# Autodesk Inventor assembly: PMax8
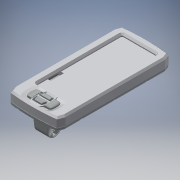
[picture p0: Inventor's stored thumbnail of the model, 180x180]
Saved by Autodesk Inventor 2018 (Build 220112000, 112)
## iProperties
Created: 2019-05-29
Part Number: PMax8
Document SubType Name: Assembly
Designer: Ash
Author: Ash
## Documents named in this file (8)
- C:\Autodesk\Skills 2019 Nationals\Competition\PMDay2\PMax8.iam
- C:\Autodesk\Skills 2019 Nationals\Competition\PMDay2\#2-KEYPAD.ipt
- C:\Autodesk\Skills 2019 Nationals\Competition\PMDay1\Front_Cover3.ipt
- C:\Autodesk\Skills 2019 Nationals\Competition\PMDay1\Display_Plate3.ipt
- C:\Autodesk\Skills 2019 Nationals\Competition\PMDay2\#4-GASKET(PMAX8).ipt
- C:\Autodesk\Skills 2019 Nationals\Competition\PMDay2\#5-BACK_COVER(PMAX8).ipt
- C:\Autodesk\Skills 2019 Nationals\Competition\PMDay2\ADDITIONAL_BUTTON.ipt
- C:\Autodesk\Skills 2019 Nationals\Competition\PMDay2\#6-SCREW.ipt
## Components (16 placed, 7 different names)
1. #2-KEYPAD:1 — Mate:6, Mate:7, Mate:8, Mate:9, Mate:11
2. Display_Plate3:1 — Mate:7, Mate:10, Mate:11
3. Front_Cover3:1 — Mate:6, Mate:8, Mate:9, Mate:10, Mate:15, Mate:16, Mate:17, Mate:18, Flush:1
4. #4-GASKET(PMAX8):1 — Mate:12, Mate:13, Mate:14, Mate:19
5. #5-BACK_COVER(PMAX8):1 — Mate:12, Mate:13, Mate:14, Mate:15, Mate:16, Mate:17, Mate:20, Mate:21, Mate:22, Mate:23, Mate:24, Mate:25, Mate:26, Mate:27, Mate:28, Mate:29, Mate:30
6. ADDITIONAL_BUTTON:1 — Mate:18, Mate:19, Flush:1
7. #6-SCREW:1 — Mate:28, Flush:2
8. #6-SCREW:2 — Mate:22, Flush:9, Flush:10
9. #6-SCREW:3 — Mate:21, Flush:8, Flush:9, Mate:30
10. #6-SCREW:4 — Mate:29, Flush:10
11. #6-SCREW:5 — Mate:23, Flush:6, Flush:7
12. #6-SCREW:6 — Mate:27, Flush:2, Flush:3
13. #6-SCREW:7 — Mate:26, Flush:3, Flush:4
14. #6-SCREW:8 — Mate:24, Flush:5, Flush:6
15. #6-SCREW:9 — Mate:25, Flush:4, Flush:5
16. #6-SCREW:10 — Mate:20, Flush:7, Flush:8
## Relationships (35: Mate 25, Flush 10)
- Mate:6 (6.35 mm): #2-KEYPAD:1 ↔ Front_Cover3:1
- Mate:7: #2-KEYPAD:1 ↔ Display_Plate3:1
- Mate:8: #2-KEYPAD:1 ↔ Front_Cover3:1
- Mate:9 (46.7868 mm): #2-KEYPAD:1 ↔ Front_Cover3:1
- Mate:10: Display_Plate3:1 ↔ Front_Cover3:1
- Mate:11: #2-KEYPAD:1 ↔ Display_Plate3:1
- Mate:12: #4-GASKET(PMAX8):1 ↔ #5-BACK_COVER(PMAX8):1
- Mate:13: #4-GASKET(PMAX8):1 ↔ #5-BACK_COVER(PMAX8):1
- Mate:14: #4-GASKET(PMAX8):1 ↔ #5-BACK_COVER(PMAX8):1
- Mate:15: Front_Cover3:1 ↔ #5-BACK_COVER(PMAX8):1
- Mate:16: Front_Cover3:1 ↔ #5-BACK_COVER(PMAX8):1
- Mate:17: Front_Cover3:1 ↔ #5-BACK_COVER(PMAX8):1
- Mate:18 (-10.16 mm): Front_Cover3:1 ↔ ADDITIONAL_BUTTON:1
- Mate:19 (6.35 mm): #4-GASKET(PMAX8):1 ↔ ADDITIONAL_BUTTON:1
- Flush:1: Front_Cover3:1 ↔ ADDITIONAL_BUTTON:1
- Mate:20: #5-BACK_COVER(PMAX8):1 ↔ #6-SCREW:10
- Mate:21: #5-BACK_COVER(PMAX8):1 ↔ #6-SCREW:3
- Mate:22: #5-BACK_COVER(PMAX8):1 ↔ #6-SCREW:2
- Mate:23: #5-BACK_COVER(PMAX8):1 ↔ #6-SCREW:5
- Mate:24: #5-BACK_COVER(PMAX8):1 ↔ #6-SCREW:8
- Mate:25: #5-BACK_COVER(PMAX8):1 ↔ #6-SCREW:9
- Mate:26: #5-BACK_COVER(PMAX8):1 ↔ #6-SCREW:7
- Mate:27: #5-BACK_COVER(PMAX8):1 ↔ #6-SCREW:6
- Mate:28: #5-BACK_COVER(PMAX8):1 ↔ #6-SCREW:1
- Mate:29: #5-BACK_COVER(PMAX8):1 ↔ #6-SCREW:4
- Flush:2: #6-SCREW:1 ↔ #6-SCREW:6
- Flush:3: #6-SCREW:6 ↔ #6-SCREW:7
- Flush:4: #6-SCREW:7 ↔ #6-SCREW:9
- Flush:5: #6-SCREW:8 ↔ #6-SCREW:9
- Flush:6: #6-SCREW:5 ↔ #6-SCREW:8
- Flush:7: #6-SCREW:5 ↔ #6-SCREW:10
- Flush:8: #6-SCREW:3 ↔ #6-SCREW:10
- Flush:9: #6-SCREW:2 ↔ #6-SCREW:3
- Flush:10: #6-SCREW:2 ↔ #6-SCREW:4
- Mate:30: #5-BACK_COVER(PMAX8):1 ↔ #6-SCREW:3
